# Autodesk Inventor assembly: Tyre
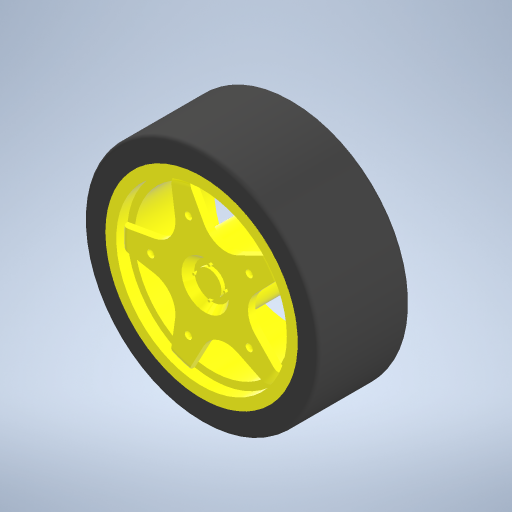
[picture p0: Inventor's stored thumbnail of the model, 512x512]
Saved by Autodesk Inventor 2023 (Build 270158000, 158)
## iProperties
Created: 2022-11-29
Part Number: Tyre
Document SubType Name: Assembly
Designer: kakik
Author: kakik
## Documents named in this file (3)
- C:\Users\kakik\Desktop\p2\Tyre.iam
- C:\Users\kakik\Desktop\p2\innertyre.ipt
- C:\Users\kakik\Desktop\p2\outertyre.ipt
## Components (2 placed, 2 different names)
1. innertyre:1 — Mate:1, Flush:1
2. outertyre:1 — Mate:1, Flush:1
## Relationships (2: Mate 1, Flush 1)
- Mate:1: innertyre:1 ↔ outertyre:1
- Flush:1: innertyre:1 ↔ outertyre:1
